# Autodesk Inventor assembly: ComputerTable
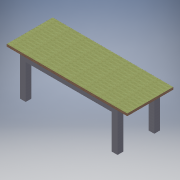
[picture p0: Inventor's stored thumbnail of the model, 180x180]
Saved by Autodesk Inventor 2017 (Build 210142000, 142)
## iProperties
Created: 2018-09-10
Part Number: ComputerTable
Document SubType Name: Assembly
Designer: emmacarlisle
Author: emmacarlisle
## Documents named in this file (3)
- \\Mac\Home\Desktop\s2-2018\ComputerTable.iam
- \\Mac\Home\Desktop\s2-2018\computerBottom.ipt
- \\Mac\Home\Desktop\s2-2018\computerTop.ipt
## Components (2 placed, 2 different names)
1. computerBottom:1 — Mate:1, Flush:1, Flush:2
2. computerTop:1 — Mate:1, Flush:1, Flush:2
## Relationships (3: Flush 2, Mate 1)
- Mate:1: computerBottom:1 ↔ computerTop:1
- Flush:1 (-200 mm): computerBottom:1 ↔ computerTop:1
- Flush:2 (-30 mm): computerBottom:1 ↔ computerTop:1
